# Autodesk Inventor assembly: NEMA 23 84mm Frame Stepper Motor
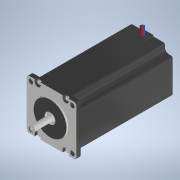
[picture p0: Inventor's stored thumbnail of the model, 180x180]
Saved by Autodesk Inventor 2021 (Build 250183000, 183)
## iProperties
Created: 2022-12-26
Part Number: NEMA 23 84mm Frame Stepper Motor
Description: FreeCAD Model
Document SubType Name: Assembly
Designer: brian
Authority: Unknown
Sending System: FreeCAD
Preprocessor: Open CASCADE STEP processor 7.6
Title: Open CASCADE Shape Model
## Documents named in this file (16)
- C:\Users\brian\Desktop\自動主席台\NEMA23\NEMA 23 84mm Frame Stepper Motor.iam
- C:\Users\brian\Desktop\自動主席台\NEMA23\Face.ipt
- C:\Users\brian\Desktop\自動主席台\NEMA23\Main Body.ipt
- C:\Users\brian\Desktop\自動主席台\NEMA23\Cap.ipt
- C:\Users\brian\Desktop\自動主席台\NEMA23\Screw 2.ipt
- C:\Users\brian\Desktop\自動主席台\NEMA23\Screw 3.ipt
- C:\Users\brian\Desktop\自動主席台\NEMA23\Screw 4.ipt
- C:\Users\brian\Desktop\自動主席台\NEMA23\Strain Relief.ipt
- C:\Users\brian\Desktop\自動主席台\NEMA23\Armature.ipt
- C:\Users\brian\Desktop\自動主席台\NEMA23\Wire - Black.ipt
- C:\Users\brian\Desktop\自動主席台\NEMA23\Screw 1.ipt
- C:\Users\brian\Desktop\自動主席台\NEMA23\Wire - Green.ipt
- C:\Users\brian\Desktop\自動主席台\NEMA23\Wire - Blue.ipt
- C:\Users\brian\Desktop\自動主席台\NEMA23\Wire - Red.ipt
- C:\Users\brian\Desktop\自動主席台\NEMA23\Face001.ipt
- C:\Users\brian\Desktop\自動主席台\NEMA23\Body020.ipt
## Components (15 placed, 15 different names)
1. 177
2. 178 — 貼合:3, 齊平:1
3. 179 — 貼合:3, 貼合:4, 齊平:1, 貼合:5, 貼合:6, 貼合:7
4. 180
5. 181
6. 182
7. 183 — 貼合:5, 貼合:6, 貼合:7, 角度:4, 相切:4, 相切:7
8. 184 — 貼合:1, 貼合:2, 貼合:4
9. 185 — 相切:1, 相切:2, 角度:2, 齊平:4
10. 186
11. 187 — 相切:1, 角度:1, 角度:2, 角度:3, 相切:5, 相切:6, 相切:7, 齊平:3, 齊平:4
12. 188 — 相切:3, 角度:1, 角度:4, 相切:4, 相切:5, 齊平:2, 齊平:3
13. 189 — 相切:2, 相切:3, 角度:3, 相切:6, 齊平:2
14. 190 — 貼合:1, 貼合:2
15. 191
## Relationships (22: Mate 7, Tangent 7, Flush 4, Angle 4)
- 貼合:1 [Mate]: 184 ↔ 190
- 貼合:2 [Mate]: 184 ↔ 190
- 貼合:3 [Mate]: 178 ↔ 179
- 貼合:4 [Mate]: 179 ↔ 184
- 齊平:1 [Flush]: 178 ↔ 179
- 貼合:5 [Mate]: 179 ↔ 183
- 貼合:6 [Mate]: 179 ↔ 183
- 貼合:7 [Mate]: 179 ↔ 183
- 相切:1 [Tangent]: 185 ↔ 187
- 相切:2 [Tangent]: 185 ↔ 189
- 相切:3 [Tangent]: 188 ↔ 189
- 角度:1 [Angle] (0 deg): 187 ↔ 188
- 角度:2 [Angle] (0 deg): 185 ↔ 187
- 角度:3 [Angle] (0 deg): 187 ↔ 189
- 角度:4 [Angle] (0 deg): 183 ↔ 188
- 相切:4 [Tangent]: 183 ↔ 188
- 相切:5 [Tangent]: 187 ↔ 188
- 相切:6 [Tangent]: 187 ↔ 189
- 相切:7 [Tangent]: 183 ↔ 187
- 齊平:2 [Flush]: 188 ↔ 189
- 齊平:3 [Flush]: 187 ↔ 188
- 齊平:4 [Flush]: 185 ↔ 187
